# Autodesk Inventor assembly: 投幣機
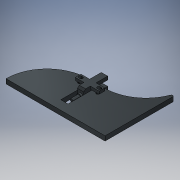
[picture p0: Inventor's stored thumbnail of the model, 180x180]
Saved by Autodesk Inventor 2017 (Build 210142000, 142)
## iProperties
Part Number: 投幣機
Material: 一般
Document SubType Name: Assembly
Designer: G
Author: G
## Documents named in this file (3)
- D:\資料\公司資料\一江資訊\投幣機\投幣機.iam
- D:\資料\公司資料\一江資訊\投幣機\D0001.ipt
- D:\資料\公司資料\一江資訊\武器把手\RX672-NW.ipt
## Components (2 placed, 2 different names)
1. D0001:1 — 貼合:2, 齊平:4, 齊平:1
2. RX672-NW:1 — 貼合:2, 齊平:4, 齊平:1
## Relationships (3: Flush 2, Mate 1)
- 貼合:2 [Mate] (0.5 mm): D0001:1 ↔ RX672-NW:1
- 齊平:4 [Flush]: D0001:1 ↔ RX672-NW:1
- 齊平:1 [Flush]: D0001:1 ↔ RX672-NW:1
